# Autodesk Inventor assembly: hipjoint1
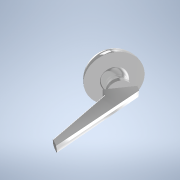
[picture p0: Inventor's stored thumbnail of the model, 180x180]
Saved by Autodesk Inventor 2021 (Build 250183000, 183)
## iProperties
Created: 2021-01-04
Part Number: hipjoint1
Document SubType Name: Assembly
Designer: USER
Author: USER
## Documents named in this file (6)
- D:\SEMESTER 5\TEKNIK REHABILITASI\PRAKTIKUM\hip joint\hipjoint1.iam
- D:\SEMESTER 5\TEKNIK REHABILITASI\PRAKTIKUM\hip joint\femortal stem.ipt
- D:\SEMESTER 5\TEKNIK REHABILITASI\PRAKTIKUM\hip joint\extraplate.ipt
- D:\SEMESTER 5\TEKNIK REHABILITASI\PRAKTIKUM\hip joint\femoral head.ipt
- D:\SEMESTER 5\TEKNIK REHABILITASI\PRAKTIKUM\hip joint\plastic liner.ipt
- D:\SEMESTER 5\TEKNIK REHABILITASI\PRAKTIKUM\hip joint\Acetabular Shell.ipt
## Components (5 placed, 5 different names)
1. femortal stem:1 — Mate:1
2. extraplate:1 — Mate:1, Insert:1
3. femoral head:1 — Insert:1, Mate:2, Ball:1
4. plastic liner:1 — Mate:2, Ball:1, Ball:2
5. Acetabular Shell:1 — Ball:2
## Relationships (5: Mate 2, BallJoint 2, Insert 1)
- Mate:1: femortal stem:1 ↔ extraplate:1
- Insert:1: extraplate:1 ↔ femoral head:1
- Mate:2: femoral head:1 ↔ plastic liner:1
- Ball:1: femoral head:1 ↔ plastic liner:1
- Ball:2: plastic liner:1 ↔ Acetabular Shell:1
